# Autodesk Inventor assembly: Vibrationsdaempfer_Einheit
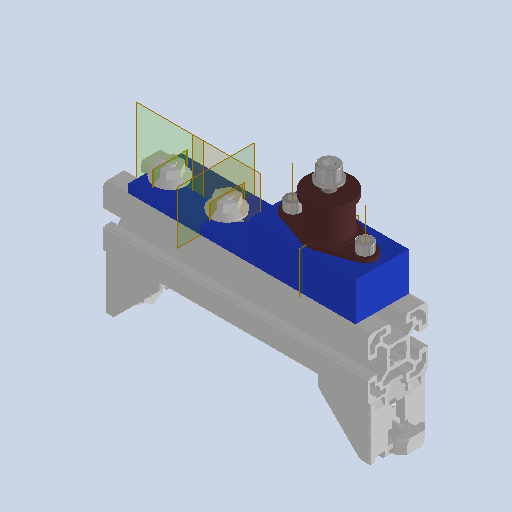
[picture p0: Inventor's stored thumbnail of the model, 512x512]
Saved by Autodesk Inventor 2025.1 (Build 291241000, 241)
## iProperties
Created: 2025-06-22
Part Number: Vibrationsdaempfer_Einheit
Document SubType Name: Assembly
Designer: Jakob
Author: Jakob
## Documents named in this file (9)
- C:\Users\Erik\Erik\Hochschule\3. Semester\CAD\CAD-Paspa\Useless Box\Eigene Bauteile\Vibrationsdaempfer\Vibrationsdaempfer_Einheit.iam
- C:\Users\Erik\Erik\Hochschule\3. Semester\CAD\CAD-Paspa\Useless Box\Eigene Bauteile\Vibrationsdaempfer\Rexroth_Profil_40x40_2175_8.ipt
- C:\Users\Erik\Erik\Hochschule\3. Semester\CAD\CAD-Paspa\Useless Box\Kaufteile\Winkel_Rexroth_40x40\Rexroth_Winkel_40x40_3D_203_MIR.iam
- C:\Users\Erik\Erik\Hochschule\3. Semester\CAD\CAD-Paspa\Useless Box\Eigene Bauteile\Vibrationsdaempfer\Adapterplatte_Vibrationsdaempfer.ipt
- C:\Users\Erik\Erik\Hochschule\3. Semester\CAD\CAD-Paspa\Useless Box\Eigene Bauteile\Vibrationsdaempfer\AIS2024\NHF19-3026-M8.ipt
- C:\Users\Erik\Erik\Hochschule\3. Semester\CAD\CAD-Paspa\Useless Box\Standart Bauteile\ISO 4762 - M6 x 12ISO.ipt
- C:\Users\Erik\Erik\Hochschule\3. Semester\CAD\CAD-Paspa\Useless Box\Standart Bauteile\ISO 4762 - M8 x 16ISO.ipt
- C:\Users\Erik\Erik\Hochschule\3. Semester\CAD\CAD-Paspa\Useless Box\Standart Bauteile\DIN 125 - A 8,4.ipt
- C:\Users\Erik\Erik\Hochschule\3. Semester\CAD\CAD-Paspa\Useless Box\Eigene Bauteile\Vibrationsdaempfer\Rexroth_Schraube_Mutter_modifiziert_fuer_daempfer.iam
## Components (11 placed, 8 different names)
1. Rexroth_Profil_40x40_2175_8:1 — Mate:1, Mate:2, Flush:1, Mate:3, Flush:3, Mate:4, Mate:6, Flush:4, Mate:10
2. Rexroth_Winkel_40x40_3D_203_MIR:1 [sub-assembly] — Mate:3, Flush:2, Flush:3
3. Rexroth_Winkel_40x40_3D_203_MIR:2 [sub-assembly] — Mate:4, Mate:5, Mate:6
4. Adapterplatte_Vibrationsdaempfer:1 — Mate:7, Flush:4, Flush:6, Mate:8, Mate:9, Mate:20, Mate:21, Angle:1, Mate:22, Mate:23, Flush:7
5. NHF19-3026-M8:1 — Flush:6, Mate:8, Mate:9, Mate:10, Mate:11, Mate:12, Mate:13, Mate:14, Mate:15, Mate:18
6. ISO 4762 - M6 x 12ISO:1 — Mate:12, Mate:14
7. ISO 4762 - M6 x 12ISO:2 — Mate:11, Mate:13
8. ISO 4762 M8 x 16:1 — Mate:15, Mate:16, Mate:17
9. DIN 125-1 A A 8,4:1 — Mate:16, Mate:17, Mate:18
10. Rexroth_Schraube_Mutter_modifiziert_fuer_daempfer:1 [sub-assembly] — Mate:22, Mate:23, Flush:7
11. Rexroth_Schraube_Mutter_modifiziert_fuer_daempfer:2 [sub-assembly] — Mate:20, Mate:21, Angle:1
## Relationships (29: Mate 22, Flush 6, Angle 1)
- Mate:1: Rexroth_Profil_40x40_2175_8:1
- Mate:2: Rexroth_Profil_40x40_2175_8:1
- Flush:1: Rexroth_Profil_40x40_2175_8:1
- Mate:3: Rexroth_Profil_40x40_2175_8:1 ↔ Rexroth_Winkel_40x40_3D_203_MIR:1
- Flush:2: Rexroth_Winkel_40x40_3D_203_MIR:1
- Flush:3: Rexroth_Profil_40x40_2175_8:1 ↔ Rexroth_Winkel_40x40_3D_203_MIR:1
- Mate:4: Rexroth_Profil_40x40_2175_8:1 ↔ Rexroth_Winkel_40x40_3D_203_MIR:2
- Mate:5: Rexroth_Winkel_40x40_3D_203_MIR:2
- Mate:6: Rexroth_Profil_40x40_2175_8:1 ↔ Rexroth_Winkel_40x40_3D_203_MIR:2
- Mate:7: Adapterplatte_Vibrationsdaempfer:1
- Flush:4: Rexroth_Profil_40x40_2175_8:1 ↔ Adapterplatte_Vibrationsdaempfer:1
- Flush:6: Adapterplatte_Vibrationsdaempfer:1 ↔ NHF19-3026-M8:1
- Mate:8: Adapterplatte_Vibrationsdaempfer:1 ↔ NHF19-3026-M8:1
- Mate:9: Adapterplatte_Vibrationsdaempfer:1 ↔ NHF19-3026-M8:1
- Mate:10 (45.642 mm): Rexroth_Profil_40x40_2175_8:1 ↔ NHF19-3026-M8:1
- Mate:11: NHF19-3026-M8:1 ↔ ISO 4762 - M6 x 12ISO:2
- Mate:12: NHF19-3026-M8:1 ↔ ISO 4762 - M6 x 12ISO:1
- Mate:13: NHF19-3026-M8:1 ↔ ISO 4762 - M6 x 12ISO:2
- Mate:14: NHF19-3026-M8:1 ↔ ISO 4762 - M6 x 12ISO:1
- Mate:15: NHF19-3026-M8:1 ↔ ISO 4762 M8 x 16:1
- Mate:16: ISO 4762 M8 x 16:1 ↔ DIN 125-1 A A 8,4:1
- Mate:17: ISO 4762 M8 x 16:1 ↔ DIN 125-1 A A 8,4:1
- Mate:18 (5.0109 mm): NHF19-3026-M8:1 ↔ DIN 125-1 A A 8,4:1
- Mate:20: Adapterplatte_Vibrationsdaempfer:1 ↔ Rexroth_Schraube_Mutter_modifiziert_fuer_daempfer:2
- Mate:21: Adapterplatte_Vibrationsdaempfer:1 ↔ Rexroth_Schraube_Mutter_modifiziert_fuer_daempfer:2
- Angle:1 (0 deg): Adapterplatte_Vibrationsdaempfer:1 ↔ Rexroth_Schraube_Mutter_modifiziert_fuer_daempfer:2
- Mate:22: Adapterplatte_Vibrationsdaempfer:1 ↔ Rexroth_Schraube_Mutter_modifiziert_fuer_daempfer:1
- Mate:23: Adapterplatte_Vibrationsdaempfer:1 ↔ Rexroth_Schraube_Mutter_modifiziert_fuer_daempfer:1
- Flush:7: Adapterplatte_Vibrationsdaempfer:1 ↔ Rexroth_Schraube_Mutter_modifiziert_fuer_daempfer:1
